# Autodesk Inventor assembly: 000.005.003 - Локоть СБ
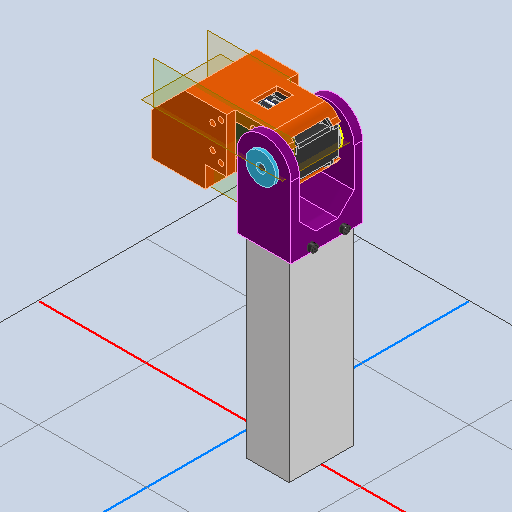
[picture p0: Inventor's stored thumbnail of the model, 512x512]
Saved by Autodesk Inventor 2022 (Build 260153000, 153)
## iProperties
Created: 2022-11-17
Part Number: 000.005.003 - Локоть СБ
Document SubType Name: Assembly
Designer: Petrov Ivan
Author: Petrov Ivan
## Documents named in this file (11)
- D:\IVAN\Ivan_desktop\Kvantorium\Projects\YouBotRobot\design\000.005.003 - Локоть СБ.iam
- D:\IVAN\Ivan_desktop\Kvantorium\Projects\YouBotRobot\design\000.005.003.001 - Основание угловое.ipt
- D:\IVAN\Ivan_desktop\Kvantorium\Projects\YouBotRobot\design\standart_components\dynamixels\mx-106\MX106T.iam
- D:\IVAN\Ivan_desktop\Kvantorium\Projects\YouBotRobot\design\000.005.003.002 - Качалка.ipt
- D:\IVAN\Ivan_desktop\Kvantorium\Projects\Autonomous_Car\Autonomous_Car\design\брус.ipt
- C:\Users\Petrov Ivan\Documents\Inventor\Content Center Files\R2022\ru-RU\ISO 4762(1)\DIN EN ISO 4762 - M2,5 x 8.ipt
- D:\IVAN\Ivan_desktop\Kvantorium\Projects\YouBotRobot\design\000.005.003.003 - Втулка.ipt
- C:\Users\Petrov Ivan\Documents\Inventor\Content Center Files\R2022\ru-RU\ISO 4762(1)\DIN EN ISO 4762 - M2,5 x 12.ipt
- C:\Users\Petrov Ivan\Documents\Inventor\Content Center Files\R2022\ru-RU\BS EN 24035\ISO 4035 - M2,5BS EN.ipt
- C:\Users\Petrov Ivan\Documents\Inventor\Content Center Files\R2022\ru-RU\BS 3692(1)\BS 3692 - M5(1).ipt
- C:\Users\Petrov Ivan\Documents\Inventor\Content Center Files\R2022\ru-RU\ISO 4762(1)\DIN EN ISO 4762 - M4 x 20.ipt
## Components (54 placed, 10 different names)
1. 000.005.003.001 - Основание угловое:1 — Совмещение:1, Заподлицо:1, Вставка:10, Вставка:11, Вставка:12, Вставка:13, Вставка:14, Вставка:15, Вставка:16, Вставка:17, Вставка:18, Вставка:19, Вставка:20, Вставка:21, Вставка:22, Вставка:23, Вставка:24, Вставка:25, Вставка:34, Вставка:35, Вставка:36, Вставка:37, Вставка:38, Вставка:39, Вставка:40, Вставка:41, Совмещение:10
2. MX106T:1 [sub-assembly] — Совмещение:1, Заподлицо:1, Совмещение:2, Совмещение:3, Совмещение:4, Совмещение:8, Совмещение:9, Вставка:26, Вставка:27, Вставка:28, Вставка:29, Вставка:30, Вставка:31, Вставка:32, Вставка:33, Совмещение:10
3. 000.005.003.002 - Качалка:1 — Совмещение:2, Совмещение:3, Совмещение:4, Совмещение:5, Совмещение:6, Совмещение:7, Вставка:1, Вставка:2, Вставка:3, Вставка:4, Вставка:5, Вставка:6, Вставка:7, Вставка:8, Вставка:42, Вставка:43, Вставка:44, Вставка:45, Вставка:46, Вставка:47, Вставка:48, Вставка:49
4. брус:1 — Совмещение:5, Совмещение:6, Совмещение:7
5. 000.005.003.003 - Втулка:1 — Совмещение:8, Совмещение:9, Вставка:9
6. BS 3692 - метрическая M5:1 — Вставка:34
7. BS 3692 - метрическая M5:2 — Вставка:35
8. BS 3692 - метрическая M5:3 — Вставка:36
9. BS 3692 - метрическая M5:4 — Вставка:37
10. DIN EN ISO 4762 M4 x 20:1 — Вставка:38
11. DIN EN ISO 4762 M4 x 20:2 — Вставка:39
12. DIN EN ISO 4762 M4 x 20:3 — Вставка:40
13. DIN EN ISO 4762 M4 x 20:4 — Вставка:41
14. BS 3692 - метрическая M5:5 — Вставка:42
15. BS 3692 - метрическая M5:6 — Вставка:43
16. BS 3692 - метрическая M5:7 — Вставка:44
17. BS 3692 - метрическая M5:8 — Вставка:45
18. DIN EN ISO 4762 M4 x 20:5 — Вставка:46
19. DIN EN ISO 4762 M4 x 20:6 — Вставка:47
20. DIN EN ISO 4762 M4 x 20:7 — Вставка:48
21. DIN EN ISO 4762 M4 x 20:8 — Вставка:49
22. DIN EN ISO 4762 M2,5 x 8:1 — Вставка:1
23. DIN EN ISO 4762 M2,5 x 8:2 — Вставка:2
24. DIN EN ISO 4762 M2,5 x 8:3 — Вставка:3
25. DIN EN ISO 4762 M2,5 x 8:4 — Вставка:4
26. DIN EN ISO 4762 M2,5 x 8:5 — Вставка:5
27. DIN EN ISO 4762 M2,5 x 8:6 — Вставка:6
28. DIN EN ISO 4762 M2,5 x 8:7 — Вставка:7
29. DIN EN ISO 4762 M2,5 x 8:8 — Вставка:8
30. DIN EN ISO 4762 M2,5 x 12:1 — Вставка:9
31. DIN EN ISO 4762 M2,5 x 8:9 — Вставка:10
32. DIN EN ISO 4762 M2,5 x 8:10 — Вставка:11
33. DIN EN ISO 4762 M2,5 x 8:11 — Вставка:12
34. DIN EN ISO 4762 M2,5 x 8:12 — Вставка:13
35. DIN EN ISO 4762 M2,5 x 8:13 — Вставка:14
36. DIN EN ISO 4762 M2,5 x 8:14 — Вставка:15
37. DIN EN ISO 4762 M2,5 x 8:15 — Вставка:16
38. DIN EN ISO 4762 M2,5 x 8:16 — Вставка:17
39. DIN EN ISO 4762 M2,5 x 8:17 — Вставка:18
40. DIN EN ISO 4762 M2,5 x 8:18 — Вставка:19
41. DIN EN ISO 4762 M2,5 x 8:19 — Вставка:20
42. DIN EN ISO 4762 M2,5 x 8:20 — Вставка:21
43. DIN EN ISO 4762 M2,5 x 8:21 — Вставка:22
44. DIN EN ISO 4762 M2,5 x 8:22 — Вставка:23
45. DIN EN ISO 4762 M2,5 x 8:23 — Вставка:24
46. DIN EN ISO 4762 M2,5 x 8:24 — Вставка:25
47. BS EN 24035 - метрическая M2,5:1 — Вставка:26
48. BS EN 24035 - метрическая M2,5:2 — Вставка:27
49. BS EN 24035 - метрическая M2,5:3 — Вставка:28
50. BS EN 24035 - метрическая M2,5:4 — Вставка:29
51. BS EN 24035 - метрическая M2,5:5 — Вставка:30
52. BS EN 24035 - метрическая M2,5:6 — Вставка:31
53. BS EN 24035 - метрическая M2,5:7 — Вставка:32
54. BS EN 24035 - метрическая M2,5:8 — Вставка:33
## Relationships (60: Insert 49, Mate 10, Flush 1)
- Совмещение:1 [Mate] (4 mm): 000.005.003.001 - Основание угловое:1 ↔ MX106T:1
- Заподлицо:1 [Flush] (8.05 mm): 000.005.003.001 - Основание угловое:1 ↔ MX106T:1
- Совмещение:2 [Mate]: MX106T:1 ↔ 000.005.003.002 - Качалка:1
- Совмещение:3 [Mate]: MX106T:1 ↔ 000.005.003.002 - Качалка:1
- Совмещение:4 [Mate]: MX106T:1 ↔ 000.005.003.002 - Качалка:1
- Совмещение:5 [Mate]: 000.005.003.002 - Качалка:1 ↔ брус:1
- Совмещение:6 [Mate] (0.25 mm): 000.005.003.002 - Качалка:1 ↔ брус:1
- Совмещение:7 [Mate] (0.25 mm): 000.005.003.002 - Качалка:1 ↔ брус:1
- Вставка:1 [Insert]: 000.005.003.002 - Качалка:1 ↔ DIN EN ISO 4762 M2,5 x 8:1
- Вставка:2 [Insert]: 000.005.003.002 - Качалка:1 ↔ DIN EN ISO 4762 M2,5 x 8:2
- Вставка:3 [Insert]: 000.005.003.002 - Качалка:1 ↔ DIN EN ISO 4762 M2,5 x 8:3
- Вставка:4 [Insert]: 000.005.003.002 - Качалка:1 ↔ DIN EN ISO 4762 M2,5 x 8:4
- Вставка:5 [Insert]: 000.005.003.002 - Качалка:1 ↔ DIN EN ISO 4762 M2,5 x 8:5
- Вставка:6 [Insert]: 000.005.003.002 - Качалка:1 ↔ DIN EN ISO 4762 M2,5 x 8:6
- Вставка:7 [Insert]: 000.005.003.002 - Качалка:1 ↔ DIN EN ISO 4762 M2,5 x 8:7
- Вставка:8 [Insert]: 000.005.003.002 - Качалка:1 ↔ DIN EN ISO 4762 M2,5 x 8:8
- Совмещение:8 [Mate]: MX106T:1 ↔ 000.005.003.003 - Втулка:1
- Совмещение:9 [Mate]: MX106T:1 ↔ 000.005.003.003 - Втулка:1
- Вставка:9 [Insert]: 000.005.003.003 - Втулка:1 ↔ DIN EN ISO 4762 M2,5 x 12:1
- Вставка:10 [Insert]: 000.005.003.001 - Основание угловое:1 ↔ DIN EN ISO 4762 M2,5 x 8:9
- Вставка:11 [Insert]: 000.005.003.001 - Основание угловое:1 ↔ DIN EN ISO 4762 M2,5 x 8:10
- Вставка:12 [Insert]: 000.005.003.001 - Основание угловое:1 ↔ DIN EN ISO 4762 M2,5 x 8:11
- Вставка:13 [Insert]: 000.005.003.001 - Основание угловое:1 ↔ DIN EN ISO 4762 M2,5 x 8:12
- Вставка:14 [Insert]: 000.005.003.001 - Основание угловое:1 ↔ DIN EN ISO 4762 M2,5 x 8:13
- Вставка:15 [Insert]: 000.005.003.001 - Основание угловое:1 ↔ DIN EN ISO 4762 M2,5 x 8:14
- Вставка:16 [Insert]: 000.005.003.001 - Основание угловое:1 ↔ DIN EN ISO 4762 M2,5 x 8:15
- Вставка:17 [Insert]: 000.005.003.001 - Основание угловое:1 ↔ DIN EN ISO 4762 M2,5 x 8:16
- Вставка:18 [Insert]: 000.005.003.001 - Основание угловое:1 ↔ DIN EN ISO 4762 M2,5 x 8:17
- Вставка:19 [Insert]: 000.005.003.001 - Основание угловое:1 ↔ DIN EN ISO 4762 M2,5 x 8:18
- Вставка:20 [Insert]: 000.005.003.001 - Основание угловое:1 ↔ DIN EN ISO 4762 M2,5 x 8:19
- Вставка:21 [Insert]: 000.005.003.001 - Основание угловое:1 ↔ DIN EN ISO 4762 M2,5 x 8:20
- Вставка:22 [Insert]: 000.005.003.001 - Основание угловое:1 ↔ DIN EN ISO 4762 M2,5 x 8:21
- Вставка:23 [Insert]: 000.005.003.001 - Основание угловое:1 ↔ DIN EN ISO 4762 M2,5 x 8:22
- Вставка:24 [Insert]: 000.005.003.001 - Основание угловое:1 ↔ DIN EN ISO 4762 M2,5 x 8:23
- Вставка:25 [Insert]: 000.005.003.001 - Основание угловое:1 ↔ DIN EN ISO 4762 M2,5 x 8:24
- Вставка:26 [Insert]: MX106T:1 ↔ BS EN 24035 - метрическая M2,5:1
- Вставка:27 [Insert]: MX106T:1 ↔ BS EN 24035 - метрическая M2,5:2
- Вставка:28 [Insert]: MX106T:1 ↔ BS EN 24035 - метрическая M2,5:3
- Вставка:29 [Insert]: MX106T:1 ↔ BS EN 24035 - метрическая M2,5:4
- Вставка:30 [Insert]: MX106T:1 ↔ BS EN 24035 - метрическая M2,5:5
- Вставка:31 [Insert]: MX106T:1 ↔ BS EN 24035 - метрическая M2,5:6
- Вставка:32 [Insert]: MX106T:1 ↔ BS EN 24035 - метрическая M2,5:7
- Вставка:33 [Insert]: MX106T:1 ↔ BS EN 24035 - метрическая M2,5:8
- Вставка:34 [Insert]: 000.005.003.001 - Основание угловое:1 ↔ BS 3692 - метрическая M5:1
- Вставка:35 [Insert]: 000.005.003.001 - Основание угловое:1 ↔ BS 3692 - метрическая M5:2
- Вставка:36 [Insert]: 000.005.003.001 - Основание угловое:1 ↔ BS 3692 - метрическая M5:3
- Вставка:37 [Insert]: 000.005.003.001 - Основание угловое:1 ↔ BS 3692 - метрическая M5:4
- Вставка:38 [Insert]: 000.005.003.001 - Основание угловое:1 ↔ DIN EN ISO 4762 M4 x 20:1
- Вставка:39 [Insert]: 000.005.003.001 - Основание угловое:1 ↔ DIN EN ISO 4762 M4 x 20:2
- Вставка:40 [Insert]: 000.005.003.001 - Основание угловое:1 ↔ DIN EN ISO 4762 M4 x 20:3
- Вставка:41 [Insert]: 000.005.003.001 - Основание угловое:1 ↔ DIN EN ISO 4762 M4 x 20:4
- Вставка:42 [Insert]: 000.005.003.002 - Качалка:1 ↔ BS 3692 - метрическая M5:5
- Вставка:43 [Insert]: 000.005.003.002 - Качалка:1 ↔ BS 3692 - метрическая M5:6
- Вставка:44 [Insert]: 000.005.003.002 - Качалка:1 ↔ BS 3692 - метрическая M5:7
- Вставка:45 [Insert]: 000.005.003.002 - Качалка:1 ↔ BS 3692 - метрическая M5:8
- Вставка:46 [Insert]: 000.005.003.002 - Качалка:1 ↔ DIN EN ISO 4762 M4 x 20:5
- Вставка:47 [Insert]: 000.005.003.002 - Качалка:1 ↔ DIN EN ISO 4762 M4 x 20:6
- Вставка:48 [Insert]: 000.005.003.002 - Качалка:1 ↔ DIN EN ISO 4762 M4 x 20:7
- Вставка:49 [Insert]: 000.005.003.002 - Качалка:1 ↔ DIN EN ISO 4762 M4 x 20:8
- Совмещение:10 [Mate]: 000.005.003.001 - Основание угловое:1 ↔ MX106T:1
